# Autodesk Inventor assembly: Body
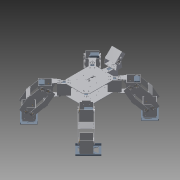
[picture p0: Inventor's stored thumbnail of the model, 180x180]
Saved by Autodesk Inventor 2013 (Build 170138000, 138)
## iProperties
Created: 2014-04-06
Document SubType Name: Assembly
Designer: andou
Author: andou
Title: Body
## Documents named in this file (6)
- C:\Users\andou\Documents\GitHub\Robotics-Project\design\RoboticsProject\project_4\Body.iam
- C:\Users\andou\Documents\GitHub\Robotics-Project\design\RoboticsProject\project_4\Bottom_Flame.ipt
- C:\Users\andou\Documents\GitHub\Robotics-Project\design\RoboticsProject\project_4\Top_Flame.ipt
- C:\Users\andou\Documents\GitHub\Robotics-Project\design\RoboticsProject\project_4\Head.iam
- C:\Users\andou\Documents\GitHub\Robotics-Project\design\RoboticsProject\project_4\Right_Leg.iam
- C:\Users\andou\Documents\GitHub\Robotics-Project\design\RoboticsProject\project_4\Left_Leg.iam
## Components (7 placed, 5 different names)
1. Bottom_Flame:1 — 挿入:1, 挿入:2, 挿入:3, 挿入:4, 挿入:5, 挿入:6, 挿入:7, 挿入:8, 挿入:9, 挿入:10
2. Top_Flame:1 — 挿入:11, 挿入:12, 挿入:13, 挿入:14, 挿入:15, 挿入:16, 挿入:17, 挿入:18, 挿入:19, 挿入:20
3. Head:1 [sub-assembly] — 挿入:9, 挿入:10, 挿入:17, 挿入:18
4. Right_Leg:1 [sub-assembly] — 挿入:2, 挿入:6, 挿入:19, 挿入:20
5. Right_Leg:2 [sub-assembly] — 挿入:1, 挿入:5, 挿入:11, 挿入:15
6. Left_Leg:1 [sub-assembly] — 挿入:4, 挿入:7, 挿入:13, 挿入:14
7. Left_Leg:2 [sub-assembly] — 挿入:3, 挿入:8, 挿入:12, 挿入:16
## Relationships (20: Insert 20)
- 挿入:1 [Insert]: Bottom_Flame:1 ↔ Right_Leg:2
- 挿入:2 [Insert]: Bottom_Flame:1 ↔ Right_Leg:1
- 挿入:3 [Insert]: Bottom_Flame:1 ↔ Left_Leg:2
- 挿入:4 [Insert]: Bottom_Flame:1 ↔ Left_Leg:1
- 挿入:5 [Insert]: Bottom_Flame:1 ↔ Right_Leg:2
- 挿入:6 [Insert]: Bottom_Flame:1 ↔ Right_Leg:1
- 挿入:7 [Insert]: Bottom_Flame:1 ↔ Left_Leg:1
- 挿入:8 [Insert]: Bottom_Flame:1 ↔ Left_Leg:2
- 挿入:9 [Insert]: Bottom_Flame:1 ↔ Head:1
- 挿入:10 [Insert]: Bottom_Flame:1 ↔ Head:1
- 挿入:11 [Insert]: Top_Flame:1 ↔ Right_Leg:2
- 挿入:12 [Insert]: Top_Flame:1 ↔ Left_Leg:2
- 挿入:13 [Insert]: Top_Flame:1 ↔ Left_Leg:1
- 挿入:14 [Insert]: Top_Flame:1 ↔ Left_Leg:1
- 挿入:15 [Insert]: Top_Flame:1 ↔ Right_Leg:2
- 挿入:16 [Insert]: Top_Flame:1 ↔ Left_Leg:2
- 挿入:17 [Insert]: Top_Flame:1 ↔ Head:1
- 挿入:18 [Insert]: Top_Flame:1 ↔ Head:1
- 挿入:19 [Insert]: Top_Flame:1 ↔ Right_Leg:1
- 挿入:20 [Insert]: Top_Flame:1 ↔ Right_Leg:1
